# Autodesk Inventor assembly: Laser
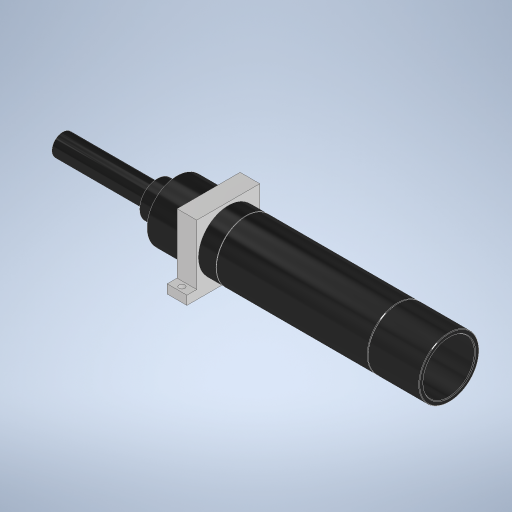
[picture p0: Inventor's stored thumbnail of the model, 512x512]
Saved by Autodesk Inventor 2023 (Build 270158000, 158)
## iProperties
Created: 2023-04-12
Part Number: Laser
Document SubType Name: Assembly
Designer: ASARe-DAQ-PC
Author: ASARe-DAQ-PC
## Documents named in this file (7)
- D:\EB camera\model of EB camera\for manufacture\Laser.iam
- D:\EB camera\model of EB camera\for manufacture\Laser body.ipt
- D:\EB camera\model of EB camera\for manufacture\Laser tube 3in.ipt
- D:\EB camera\model of EB camera\for manufacture\Laser tube.ipt
- D:\EB camera\model of EB camera\for manufacture\Laser tube3.ipt
- D:\EB camera\model of EB camera\for manufacture\Laser tube4.ipt
- D:\EB camera\model of EB camera\for manufacture\Laser holder3.ipt
## Components (6 placed, 6 different names)
1. Laser body:1 — Mate:4, Insert:3
2. Laser tube 3in:1 — Insert:1
3. Laser tube:1 — Insert:1, Mate:1, Mate:2, Mate:4
4. Laser tube3:1 — Mate:1, Mate:2, Insert:4
5. Laser tube4:1 — Insert:3, Insert:5
6. Laser holder3:1 — Insert:4, Insert:5
## Relationships (7: Insert 4, Mate 3)
- Insert:1: Laser tube 3in:1 ↔ Laser tube:1
- Mate:1: Laser tube:1 ↔ Laser tube3:1
- Mate:2: Laser tube:1 ↔ Laser tube3:1
- Mate:4: Laser body:1 ↔ Laser tube:1
- Insert:3: Laser body:1 ↔ Laser tube4:1
- Insert:4: Laser tube3:1 ↔ Laser holder3:1
- Insert:5: Laser tube4:1 ↔ Laser holder3:1
